# Autodesk Inventor assembly: pto-chain
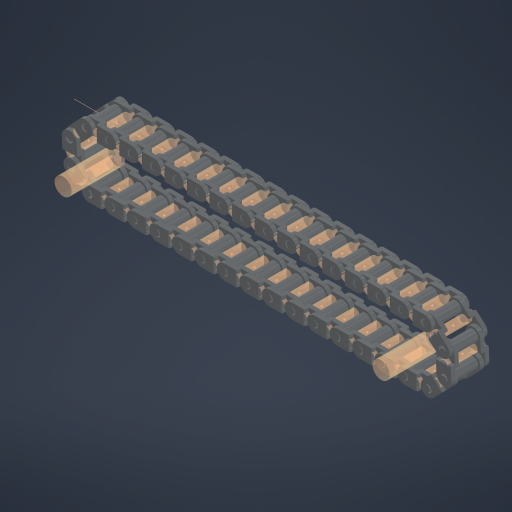
[picture p0: Inventor's stored thumbnail of the model, 512x512]
Saved by Autodesk Inventor 2023.2 (Build 272271000, 271)
## iProperties
RuleStatus: InUse
Created: 2020-07-07
Part Number: pto-chain
Document SubType Name: Assembly
Designer: yuany
AfterDocOpen0: Open Form
Author: yuany
## Documents named in this file (3)
- D:\CAD\Parts\custom\vex\pto-chain.iam
- D:\CAD\Parts\standard\Motion\Chain\Reference parts\Workpoint Pattern.ipt
- D:\CAD\Parts\standard\Motion\Chain\Reference parts\Chain.ipt
## Components (37 placed, 2 different names)
1. Workpoint Pattern:1 — Mate:4, Mate:5, Angle:1
2. Chain:1 — Mate:4, Mate:5, Angle:1
3. Chain:2
4. Chain:3
5. Chain:4
6. Chain:5
7. Chain:6
8. Chain:7
9. Chain:8
10. Chain:9
11. Chain:10
12. Chain:11
13. Chain:12
14. Chain:13
15. Chain:14
16. Chain:15
17. Chain:16
18. Chain:17
19. Chain:18
20. Chain:19
21. Chain:20
22. Chain:21
23. Chain:22
24. Chain:23
25. Chain:24
26. Chain:25
27. Chain:26
28. Chain:27
29. Chain:28
30. Chain:29
31. Chain:30
32. Chain:31
33. Chain:32
34. Chain:33
35. Chain:34
36. Chain:35
37. Chain:36
## Component patterns: (36 elements, first: Chain:1)
## Relationships (3: Mate 2, Angle 1)
- Mate:4: Workpoint Pattern:1 ↔ Chain:1
- Mate:5: Workpoint Pattern:1 ↔ Chain:1
- Angle:1 (180 deg): Workpoint Pattern:1 ↔ Chain:1
## Named parameters: Center_Distance = 94.5196 mm, Sprocket1 = 16.59335 mm, Sprocket2 = 16.59335 mm, CenterDistance = 94.5196 mm
